# Autodesk Inventor assembly: Carriage_Assembly
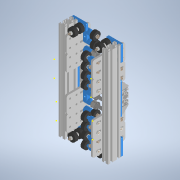
[picture p0: Inventor's stored thumbnail of the model, 180x180]
Saved by Autodesk Inventor 2021 (Build 250183000, 183)
## iProperties
Created: 2021-09-08
Part Number: Carriage_Assembly
Document SubType Name: Assembly
Designer: Jorian Brusind
Author: Jorian Brusind
## Documents named in this file (18)
- C:\Users\Jorian Brusind\Documents\GitHub\HyperRail\Inventor Files\Carriage_Assembly.iam
- C:\Users\Jorian Brusind\Documents\GitHub\HyperRail\Inventor Files\8020_Sets\IPT_20_Series\IPT_20_Series\20-2040_150mm.ipt
- C:\Users\Jorian Brusind\Documents\GitHub\HyperRail\Inventor Files\X_CarriageR_V2_0.iam
- C:\Users\Jorian Brusind\Documents\GitHub\HyperRail\Inventor Files\X_Carriage_V2_0.iam
- C:\Users\Jorian Brusind\Documents\GitHub\HyperRail\Inventor Files\8020_Sets\IPT_20_Series\Extra_20_Series\8020_14056m\14056_m.ipt
- C:\Users\Jorian Brusind\Documents\GitHub\HyperRail\Inventor Files\Buffer.iam
- C:\Users\Jorian Brusind\Documents\GitHub\HyperRail\Inventor Files\Metric Spacer_Standoffs\hex spacer standoff nut M5 L30.ipt
- C:\Users\Jorian Brusind\Documents\GitHub\HyperRail\Inventor Files\Carriage_Horizontal_Spacer.ipt
- C:\Users\Jorian Brusind\Documents\GitHub\HyperRail\Inventor Files\8020_Sets\IPT_20_Series\IPT_20_Series\20-2040_400mm.ipt
- C:\Users\Jorian Brusind\Documents\GitHub\HyperRail\Inventor Files\X_CarriageL_V2_1_Short.iam
- C:\Users\Jorian Brusind\Documents\GitHub\HyperRail\Inventor Files\X_CarriageR_V2_1_Short.iam
- C:\Users\Jorian Brusind\Documents\GitHub\HyperRail\Inventor Files\Buffer_L.iam
- C:\Users\Jorian Brusind\Documents\GitHub\HyperRail\Inventor Files\Metric bolt\Bolt M5 45mm.ipt
- C:\Users\Jorian Brusind\Documents\GitHub\HyperRail\Inventor Files\Metric bolt\Bolt M5 10mm.ipt
- C:\Users\Jorian Brusind\Documents\GitHub\HyperRail\Inventor Files\Metric nuts\Nut M5.ipt
- C:\Users\Jorian Brusind\Documents\GitHub\HyperRail\Inventor Files\X_CarriageL_V2_0_Short.iam
- C:\Users\Jorian Brusind\Documents\GitHub\HyperRail\Inventor Files\X_CarriageR_V2_0_Short.iam
- C:\Users\Jorian Brusind\Documents\GitHub\HyperRail\Inventor Files\din-508-t-slot-nut-t-nut-m4-m42-2.snapshot.3\STEPS\DIN 508, T-Slot Nut M5.ipt
## Components (98 placed, 17 different names)
1. 20-2040_150mm:1 — Mate:20, Mate:21, Mate:22, Mate:23, Mate:80, Flush:33, Flush:94, Flush:96, Flush:99, Flush:102, Flush:114
2. X_CarriageR_V2_0:1 [sub-assembly] — Mate:96, Flush:56, Flush:63, Flush:65, Flush:67, Mate:124, Mate:126, Mate:127, Mate:134, Mate:143, Mate:144, Mate:145, Mate:146, Mate:181, Mate:182, Mate:183, Mate:184, Flush:82, Flush:83, Flush:84, Mate:278
3. 14056_m:1 — Mate:21, Flush:26, Flush:38, Mate:167, Mate:168, Mate:169, Mate:170
4. 14056_m:2 — Mate:20, Flush:26, Mate:70, Flush:37, Flush:39, Mate:163, Mate:164, Mate:165, Mate:166
5. 14056_m:3 — Mate:22, Flush:13, Mate:155, Mate:156, Mate:157, Mate:158, Flush:115
6. 14056_m:4 — Mate:23, Flush:13, Mate:72, Mate:159, Mate:160, Mate:161, Mate:162, Flush:114, Flush:115, Flush:116
7. Buffer:2 [sub-assembly] — Mate:86, Flush:55, Mate:202, Mate:203, Mate:206, Mate:207, Flush:120
8. Buffer:3 [sub-assembly] — Flush:42, Mate:87, Mate:196, Mate:197, Mate:198, Mate:199, Flush:119, Mate:281
9. Carriage_Horizontal_Spacer:1 — Mate:72, Mate:79, Mate:80, Flush:116, Flush:117
10. Carriage_Horizontal_Spacer:2 — Mate:70, Mate:84, Flush:37, Flush:38, Flush:117
11. 20-2040_400mm:1 — Flush:30, Mate:75, Mate:76, Mate:79, Flush:33, Flush:36, Mate:86, Flush:55, Mate:111, Mate:112, Flush:59, Mate:140, Flush:71, Mate:216, Mate:217, Flush:97, Flush:98, Flush:100, Flush:101, Flush:103, Flush:104, Flush:118, Flush:120
12. 20-2040_400mm:2 — Flush:30, Flush:36, Mate:84, Flush:39, Flush:42, Mate:87, Mate:96, Mate:107, Mate:139, Flush:70, Mate:211, Mate:213, Mate:219, Mate:221, Mate:223, Flush:92, Flush:93, Flush:95, Flush:119, Flush:121
13. X_Carriage_V2_0:2 [sub-assembly] — Mate:107, Flush:63, Flush:64, Flush:65, Flush:67, Mate:130, Mate:131, Mate:138, Mate:152, Mate:153, Mate:154, Mate:179, Mate:180, Mate:185, Mate:186, Mate:191, Flush:81, Flush:90, Flush:91, Mate:277
14. X_CarriageL_V2_1_Short:1 [sub-assembly] — Mate:112, Flush:57, Flush:66, Mate:132, Mate:133, Mate:141, Mate:142, Mate:147, Mate:148, Flush:87, Mate:279
15. X_CarriageR_V2_1_Short:1 [sub-assembly] — Mate:111, Flush:56, Flush:57, Flush:59, Flush:64, Flush:66, Mate:135, Mate:136, Mate:137, Mate:149, Mate:150, Mate:151, Flush:86, Flush:112, Mate:276
16. hex spacer standoff nut M5 L30:1 — Mate:124, Mate:126, Mate:133
17. hex spacer standoff nut M5 L30:2 — Mate:130, Mate:135
18. hex spacer standoff nut M5 L30:3 — Mate:127, Mate:132, Mate:134
19. hex spacer standoff nut M5 L30:4 — Mate:131, Mate:136, Mate:137, Mate:138
20. Buffer_L:1 [sub-assembly] — Mate:139, Flush:70, Mate:192, Mate:193, Mate:194, Mate:195, Flush:121, Mate:280
21. Buffer_L:2 [sub-assembly] — Mate:140, Flush:71, Mate:200, Mate:201, Mate:204, Mate:205, Flush:118
22. Bolt M5 45mm:1 — Mate:142, Mate:148
23. Bolt M5 45mm:2 — Mate:141, Mate:147
24. Bolt M5 45mm:3 — Mate:143, Mate:145
25. Bolt M5 45mm:4 — Mate:144, Mate:146
26. Bolt M5 45mm:5 — Mate:150, Flush:73
27. Bolt M5 45mm:6 — Mate:149, Flush:73, Mate:151
28. Bolt M5 45mm:7 — Mate:153, Flush:74
29. Bolt M5 45mm:8 — Mate:152, Flush:74, Mate:154
30. Bolt M5 10mm:1 — Mate:156, Mate:158, Mate:231
31. Bolt M5 10mm:2 — Mate:155, Mate:157, Mate:232
32. Bolt M5 10mm:3 — Mate:164, Mate:165, Mate:227
33. Bolt M5 10mm:4 — Mate:168, Mate:169, Mate:222
34. Bolt M5 10mm:5 — Mate:163, Mate:166, Mate:228
35. Bolt M5 10mm:6 — Mate:167, Mate:170, Mate:224
36. Bolt M5 10mm:7 — Mate:160, Mate:162, Mate:234
37. Bolt M5 10mm:8 — Mate:159, Mate:161, Mate:233
38. Bolt M5 45mm:9 — Mate:181, Mate:183, Mate:187
39. Bolt M5 45mm:10 — Mate:182, Mate:184, Mate:188
40. Bolt M5 45mm:11 — Mate:179, Mate:185, Mate:189
41. Bolt M5 45mm:12 — Mate:180, Mate:186, Mate:190
42. Nut M5:5 — Mate:187, Flush:77
43. Nut M5:6 — Mate:188, Flush:76, Flush:77
44. Nut M5:7 — Mate:189, Flush:75
45. Nut M5:8 — Mate:190, Flush:75, Flush:76, Mate:191
46. Bolt M5 10mm:9 — Mate:192, Mate:195, Mate:225
47. Bolt M5 10mm:10 — Mate:193, Mate:194, Mate:226
48. Bolt M5 10mm:11 — Mate:202, Mate:206, Mate:230
49. Bolt M5 10mm:12 — Mate:201, Mate:205, Mate:236
50. Bolt M5 10mm:13 — Mate:203, Mate:207, Mate:229
51. Bolt M5 10mm:14 — Mate:200, Mate:204, Mate:235
52. Bolt M5 10mm:15 — Mate:197, Mate:198
53. Bolt M5 10mm:16 — Mate:196, Mate:199, Mate:220
54. X_Carriage_V2_0:3 [sub-assembly] — Mate:211, Flush:81, Flush:90, Flush:91, Mate:249, Mate:250, Mate:251, Mate:252, Mate:253, Mate:254, Mate:255, Mate:256, Mate:277, Mate:280
55. X_CarriageR_V2_0:2 [sub-assembly] — Flush:82, Mate:213, Flush:83, Flush:84, Mate:237, Mate:238, Mate:239, Mate:240, Mate:257, Mate:258, Mate:259, Mate:260, Mate:269, Mate:278, Mate:281
56. X_CarriageL_V2_0_Short:1 [sub-assembly] — Mate:217, Flush:87, Mate:241, Mate:242, Mate:243, Mate:244, Mate:270, Flush:113, Mate:279
57. X_CarriageR_V2_0_Short:1 [sub-assembly] — Flush:86, Mate:216, Mate:245, Mate:246, Mate:247, Mate:248, Flush:112, Flush:113, Mate:276
58. DIN 508, T-Slot Nut M5:1 — Mate:220, Mate:221
59. DIN 508, T-Slot Nut M5:2 — Mate:222, Mate:223
60. DIN 508, T-Slot Nut M5:3 — Mate:219
61. DIN 508, T-Slot Nut M5:4 — Mate:225, Flush:93
62. DIN 508, T-Slot Nut M5:5 — Mate:226, Flush:92
63. DIN 508, T-Slot Nut M5:6 — Mate:227, Flush:96
64. DIN 508, T-Slot Nut M5:7 — Mate:224, Flush:94
65. DIN 508, T-Slot Nut M5:8 — Mate:228, Flush:95
66. DIN 508, T-Slot Nut M5:10 — Mate:229, Flush:98
67. DIN 508, T-Slot Nut M5:11 — Mate:230, Flush:97
68. DIN 508, T-Slot Nut M5:12 — Mate:232, Flush:100
69. DIN 508, T-Slot Nut M5:13 — Mate:231, Flush:99
70. DIN 508, T-Slot Nut M5:14 — Mate:233, Flush:102
71. DIN 508, T-Slot Nut M5:15 — Mate:234, Flush:101
72. DIN 508, T-Slot Nut M5:16 — Mate:235, Flush:103
73. DIN 508, T-Slot Nut M5:17 — Mate:236, Flush:104
74. Bolt M5 45mm:13 — Mate:238, Mate:240, Mate:265
75. Bolt M5 45mm:14 — Mate:237, Mate:239, Mate:266
76. Bolt M5 45mm:15 — Mate:241, Mate:244, Mate:261
77. Bolt M5 45mm:16 — Mate:242, Mate:243, Mate:262
78. Bolt M5 45mm:17 — Mate:251, Mate:252, Mate:274
79. Bolt M5 45mm:18 — Mate:245, Mate:246, Mate:264, Mate:275
80. Bolt M5 45mm:19 — Mate:249, Mate:250, Mate:273
81. Bolt M5 45mm:20 — Mate:247, Mate:248, Mate:263
82. Bolt M5 45mm:21 — Mate:253, Mate:255, Mate:271
83. Bolt M5 45mm:22 — Mate:254, Mate:256, Mate:272
84. Bolt M5 45mm:23 — Mate:257, Mate:260, Mate:267
85. Bolt M5 45mm:24 — Mate:258, Mate:259, Mate:268
86. Nut M5:9 — Mate:264
87. Nut M5:10 — Mate:262, Flush:106, Mate:270
88. Nut M5:11 — Mate:266, Flush:105, Mate:269, Flush:110
89. Nut M5:12 — Mate:265, Flush:105
90. Nut M5:13 — Mate:267
91. Nut M5:14 — Mate:268, Flush:109
92. Nut M5:15 — Mate:263, Flush:111
93. Nut M5:16 — Mate:261, Flush:106
94. Nut M5:17 — Mate:274
95. Nut M5:18 — Mate:273, Flush:110
96. Nut M5:19 — Mate:271, Flush:109
97. Nut M5:20 — Mate:272
98. Nut M5:21 — Mate:275, Flush:111
## Relationships (220: Mate 157, Flush 63)
- Mate:20 (3 mm): 20-2040_150mm:1 ↔ 14056_m:2
- Mate:21 (3 mm): 20-2040_150mm:1 ↔ 14056_m:1
- Mate:22 (3 mm): 20-2040_150mm:1 ↔ 14056_m:3
- Mate:23 (3 mm): 20-2040_150mm:1 ↔ 14056_m:4
- Flush:13: 14056_m:3 ↔ 14056_m:4
- Flush:26: 14056_m:1 ↔ 14056_m:2
- Mate:70: 14056_m:2 ↔ Carriage_Horizontal_Spacer:2
- Mate:72: 14056_m:4 ↔ Carriage_Horizontal_Spacer:1
- Flush:30: 20-2040_400mm:1 ↔ 20-2040_400mm:2
- Mate:75: 20-2040_400mm:1
- Mate:76: 20-2040_400mm:1
- Mate:79: Carriage_Horizontal_Spacer:1 ↔ 20-2040_400mm:1
- Mate:80: 20-2040_150mm:1 ↔ Carriage_Horizontal_Spacer:1
- Flush:33: 20-2040_150mm:1 ↔ 20-2040_400mm:1
- Flush:36: 20-2040_400mm:1 ↔ 20-2040_400mm:2
- Mate:84: Carriage_Horizontal_Spacer:2 ↔ 20-2040_400mm:2
- Flush:37: 14056_m:2 ↔ Carriage_Horizontal_Spacer:2
- Flush:38: 14056_m:1 ↔ Carriage_Horizontal_Spacer:2
- Flush:39: 14056_m:2 ↔ 20-2040_400mm:2
- Mate:86: Buffer:2 ↔ 20-2040_400mm:1
- Flush:42: Buffer:3 ↔ 20-2040_400mm:2
- Mate:87: Buffer:3 ↔ 20-2040_400mm:2
- Mate:96: X_CarriageR_V2_0:1 ↔ 20-2040_400mm:2
- Flush:55: Buffer:2 ↔ 20-2040_400mm:1
- Mate:107: 20-2040_400mm:2 ↔ X_Carriage_V2_0:2
- Mate:111: 20-2040_400mm:1 ↔ X_CarriageR_V2_1_Short:1
- Flush:56: X_CarriageR_V2_0:1 ↔ X_CarriageR_V2_1_Short:1
- Mate:112: 20-2040_400mm:1 ↔ X_CarriageL_V2_1_Short:1
- Flush:57: X_CarriageL_V2_1_Short:1 ↔ X_CarriageR_V2_1_Short:1
- Flush:59: 20-2040_400mm:1 ↔ X_CarriageR_V2_1_Short:1
- Flush:63: X_CarriageR_V2_0:1 ↔ X_Carriage_V2_0:2
- Flush:64: X_Carriage_V2_0:2 ↔ X_CarriageR_V2_1_Short:1
- Flush:65: X_CarriageR_V2_0:1 ↔ X_Carriage_V2_0:2
- Flush:66: X_CarriageL_V2_1_Short:1 ↔ X_CarriageR_V2_1_Short:1
- Flush:67: X_CarriageR_V2_0:1 ↔ X_Carriage_V2_0:2
- Mate:124: X_CarriageR_V2_0:1 ↔ hex spacer standoff nut M5 L30:1
- Mate:126: X_CarriageR_V2_0:1 ↔ hex spacer standoff nut M5 L30:1
- Mate:127: X_CarriageR_V2_0:1 ↔ hex spacer standoff nut M5 L30:3
- Mate:130: X_Carriage_V2_0:2 ↔ hex spacer standoff nut M5 L30:2
- Mate:131: X_Carriage_V2_0:2 ↔ hex spacer standoff nut M5 L30:4
- Mate:132: X_CarriageL_V2_1_Short:1 ↔ hex spacer standoff nut M5 L30:3
- Mate:133: X_CarriageL_V2_1_Short:1 ↔ hex spacer standoff nut M5 L30:1
- Mate:134: X_CarriageR_V2_0:1 ↔ hex spacer standoff nut M5 L30:3
- Mate:135: X_CarriageR_V2_1_Short:1 ↔ hex spacer standoff nut M5 L30:2
- Mate:136: X_CarriageR_V2_1_Short:1 ↔ hex spacer standoff nut M5 L30:4
- Mate:137: X_CarriageR_V2_1_Short:1 ↔ hex spacer standoff nut M5 L30:4
- Mate:138: X_Carriage_V2_0:2 ↔ hex spacer standoff nut M5 L30:4
- Mate:139: 20-2040_400mm:2 ↔ Buffer_L:1
- Flush:70: 20-2040_400mm:2 ↔ Buffer_L:1
- Mate:140: 20-2040_400mm:1 ↔ Buffer_L:2
- Flush:71: 20-2040_400mm:1 ↔ Buffer_L:2
- Mate:141: X_CarriageL_V2_1_Short:1 ↔ Bolt M5 45mm:2
- Mate:142: X_CarriageL_V2_1_Short:1 ↔ Bolt M5 45mm:1
- Mate:143: X_CarriageR_V2_0:1 ↔ Bolt M5 45mm:3
- Mate:144: X_CarriageR_V2_0:1 ↔ Bolt M5 45mm:4
- Mate:145: X_CarriageR_V2_0:1 ↔ Bolt M5 45mm:3
- Mate:146: X_CarriageR_V2_0:1 ↔ Bolt M5 45mm:4
- Mate:147: X_CarriageL_V2_1_Short:1 ↔ Bolt M5 45mm:2
- Mate:148: X_CarriageL_V2_1_Short:1 ↔ Bolt M5 45mm:1
- Mate:149: X_CarriageR_V2_1_Short:1 ↔ Bolt M5 45mm:6
- Mate:150: X_CarriageR_V2_1_Short:1 ↔ Bolt M5 45mm:5
- Flush:73: Bolt M5 45mm:5 ↔ Bolt M5 45mm:6
- Mate:151: X_CarriageR_V2_1_Short:1 ↔ Bolt M5 45mm:6
- Mate:152: X_Carriage_V2_0:2 ↔ Bolt M5 45mm:8
- Mate:153: X_Carriage_V2_0:2 ↔ Bolt M5 45mm:7
- Flush:74: Bolt M5 45mm:7 ↔ Bolt M5 45mm:8
- Mate:154: X_Carriage_V2_0:2 ↔ Bolt M5 45mm:8
- Mate:155: 14056_m:3 ↔ Bolt M5 10mm:2
- Mate:156: 14056_m:3 ↔ Bolt M5 10mm:1
- Mate:157: 14056_m:3 ↔ Bolt M5 10mm:2
- Mate:158: 14056_m:3 ↔ Bolt M5 10mm:1
- Mate:159: 14056_m:4 ↔ Bolt M5 10mm:8
- Mate:160: 14056_m:4 ↔ Bolt M5 10mm:7
- Mate:161: 14056_m:4 ↔ Bolt M5 10mm:8
- Mate:162: 14056_m:4 ↔ Bolt M5 10mm:7
- Mate:163: 14056_m:2 ↔ Bolt M5 10mm:5
- Mate:164: 14056_m:2 ↔ Bolt M5 10mm:3
- Mate:165: 14056_m:2 ↔ Bolt M5 10mm:3
- Mate:166: 14056_m:2 ↔ Bolt M5 10mm:5
- Mate:167: 14056_m:1 ↔ Bolt M5 10mm:6
- Mate:168: 14056_m:1 ↔ Bolt M5 10mm:4
- Mate:169: 14056_m:1 ↔ Bolt M5 10mm:4
- Mate:170: 14056_m:1 ↔ Bolt M5 10mm:6
- Mate:179: X_Carriage_V2_0:2 ↔ Bolt M5 45mm:11
- Mate:180: X_Carriage_V2_0:2 ↔ Bolt M5 45mm:12
- Mate:181: X_CarriageR_V2_0:1 ↔ Bolt M5 45mm:9
- Mate:182: X_CarriageR_V2_0:1 ↔ Bolt M5 45mm:10
- Mate:183: X_CarriageR_V2_0:1 ↔ Bolt M5 45mm:9
- Mate:184: X_CarriageR_V2_0:1 ↔ Bolt M5 45mm:10
- Mate:185: X_Carriage_V2_0:2 ↔ Bolt M5 45mm:11
- Mate:186: X_Carriage_V2_0:2 ↔ Bolt M5 45mm:12
- Mate:187: Bolt M5 45mm:9 ↔ Nut M5:5
- Mate:188: Bolt M5 45mm:10 ↔ Nut M5:6
- Mate:189: Bolt M5 45mm:11 ↔ Nut M5:7
- Mate:190: Bolt M5 45mm:12 ↔ Nut M5:8
- Flush:75: Nut M5:7 ↔ Nut M5:8
- Flush:76: Nut M5:6 ↔ Nut M5:8
- Flush:77: Nut M5:5 ↔ Nut M5:6
- Mate:191: X_Carriage_V2_0:2 ↔ Nut M5:8
- Mate:192: Buffer_L:1 ↔ Bolt M5 10mm:9
- Mate:193: Buffer_L:1 ↔ Bolt M5 10mm:10
- Mate:194: Buffer_L:1 ↔ Bolt M5 10mm:10
- Mate:195: Buffer_L:1 ↔ Bolt M5 10mm:9
- Mate:196: Buffer:3 ↔ Bolt M5 10mm:16
- Mate:197: Buffer:3 ↔ Bolt M5 10mm:15
- Mate:198: Buffer:3 ↔ Bolt M5 10mm:15
- Mate:199: Buffer:3 ↔ Bolt M5 10mm:16
- Mate:200: Buffer_L:2 ↔ Bolt M5 10mm:14
- Mate:201: Buffer_L:2 ↔ Bolt M5 10mm:12
- Mate:202: Buffer:2 ↔ Bolt M5 10mm:11
- Mate:203: Buffer:2 ↔ Bolt M5 10mm:13
- Mate:204: Buffer_L:2 ↔ Bolt M5 10mm:14
- Mate:205: Buffer_L:2 ↔ Bolt M5 10mm:12
- Mate:206: Buffer:2 ↔ Bolt M5 10mm:11
- Mate:207: Buffer:2 ↔ Bolt M5 10mm:13
- Mate:211: 20-2040_400mm:2 ↔ X_Carriage_V2_0:3
- Flush:81: X_Carriage_V2_0:2 ↔ X_Carriage_V2_0:3
- Flush:82: X_CarriageR_V2_0:1 ↔ X_CarriageR_V2_0:2
- Mate:213: 20-2040_400mm:2 ↔ X_CarriageR_V2_0:2
- Flush:83: X_CarriageR_V2_0:1 ↔ X_CarriageR_V2_0:2
- Flush:84: X_CarriageR_V2_0:1 ↔ X_CarriageR_V2_0:2
- Flush:86: X_CarriageR_V2_1_Short:1 ↔ X_CarriageR_V2_0_Short:1
- Mate:216: 20-2040_400mm:1 ↔ X_CarriageR_V2_0_Short:1
- Mate:217: 20-2040_400mm:1 ↔ X_CarriageL_V2_0_Short:1
- Flush:87: X_CarriageL_V2_1_Short:1 ↔ X_CarriageL_V2_0_Short:1
- Flush:90: X_Carriage_V2_0:2 ↔ X_Carriage_V2_0:3
- Flush:91: X_Carriage_V2_0:2 ↔ X_Carriage_V2_0:3
- Mate:219: 20-2040_400mm:2 ↔ DIN 508, T-Slot Nut M5:3
- Mate:220: Bolt M5 10mm:16 ↔ DIN 508, T-Slot Nut M5:1
- Mate:221: 20-2040_400mm:2 ↔ DIN 508, T-Slot Nut M5:1
- Mate:222: Bolt M5 10mm:4 ↔ DIN 508, T-Slot Nut M5:2
- Mate:223: 20-2040_400mm:2 ↔ DIN 508, T-Slot Nut M5:2
- Mate:224: Bolt M5 10mm:6 ↔ DIN 508, T-Slot Nut M5:7
- Mate:225: Bolt M5 10mm:9 ↔ DIN 508, T-Slot Nut M5:4
- Mate:226: Bolt M5 10mm:10 ↔ DIN 508, T-Slot Nut M5:5
- Flush:92: 20-2040_400mm:2 ↔ DIN 508, T-Slot Nut M5:5
- Flush:93: 20-2040_400mm:2 ↔ DIN 508, T-Slot Nut M5:4
- Flush:94: 20-2040_150mm:1 ↔ DIN 508, T-Slot Nut M5:7
- Mate:227: Bolt M5 10mm:3 ↔ DIN 508, T-Slot Nut M5:6
- Mate:228: Bolt M5 10mm:5 ↔ DIN 508, T-Slot Nut M5:8
- Flush:95: 20-2040_400mm:2 ↔ DIN 508, T-Slot Nut M5:8
- Flush:96: 20-2040_150mm:1 ↔ DIN 508, T-Slot Nut M5:6
- Mate:229: Bolt M5 10mm:13 ↔ DIN 508, T-Slot Nut M5:10
- Mate:230: Bolt M5 10mm:11 ↔ DIN 508, T-Slot Nut M5:11
- Flush:97: 20-2040_400mm:1 ↔ DIN 508, T-Slot Nut M5:11
- Flush:98: 20-2040_400mm:1 ↔ DIN 508, T-Slot Nut M5:10
- Mate:231: Bolt M5 10mm:1 ↔ DIN 508, T-Slot Nut M5:13
- Mate:232: Bolt M5 10mm:2 ↔ DIN 508, T-Slot Nut M5:12
- Flush:99: 20-2040_150mm:1 ↔ DIN 508, T-Slot Nut M5:13
- Flush:100: 20-2040_400mm:1 ↔ DIN 508, T-Slot Nut M5:12
- Mate:233: Bolt M5 10mm:8 ↔ DIN 508, T-Slot Nut M5:14
- Mate:234: Bolt M5 10mm:7 ↔ DIN 508, T-Slot Nut M5:15
- Flush:101: 20-2040_400mm:1 ↔ DIN 508, T-Slot Nut M5:15
- Flush:102: 20-2040_150mm:1 ↔ DIN 508, T-Slot Nut M5:14
- Mate:235: Bolt M5 10mm:14 ↔ DIN 508, T-Slot Nut M5:16
- Flush:103: 20-2040_400mm:1 ↔ DIN 508, T-Slot Nut M5:16
- Mate:236: Bolt M5 10mm:12 ↔ DIN 508, T-Slot Nut M5:17
- Flush:104: 20-2040_400mm:1 ↔ DIN 508, T-Slot Nut M5:17
- Mate:237: X_CarriageR_V2_0:2 ↔ Bolt M5 45mm:14
- Mate:238: X_CarriageR_V2_0:2 ↔ Bolt M5 45mm:13
- Mate:239: X_CarriageR_V2_0:2 ↔ Bolt M5 45mm:14
- Mate:240: X_CarriageR_V2_0:2 ↔ Bolt M5 45mm:13
- Mate:241: X_CarriageL_V2_0_Short:1 ↔ Bolt M5 45mm:15
- Mate:242: X_CarriageL_V2_0_Short:1 ↔ Bolt M5 45mm:16
- Mate:243: X_CarriageL_V2_0_Short:1 ↔ Bolt M5 45mm:16
- Mate:244: X_CarriageL_V2_0_Short:1 ↔ Bolt M5 45mm:15
- Mate:245: X_CarriageR_V2_0_Short:1 ↔ Bolt M5 45mm:18
- Mate:246: X_CarriageR_V2_0_Short:1 ↔ Bolt M5 45mm:18
- Mate:247: X_CarriageR_V2_0_Short:1 ↔ Bolt M5 45mm:20
- Mate:248: X_CarriageR_V2_0_Short:1 ↔ Bolt M5 45mm:20
- Mate:249: X_Carriage_V2_0:3 ↔ Bolt M5 45mm:19
- Mate:250: X_Carriage_V2_0:3 ↔ Bolt M5 45mm:19
- Mate:251: X_Carriage_V2_0:3 ↔ Bolt M5 45mm:17
- Mate:252: X_Carriage_V2_0:3 ↔ Bolt M5 45mm:17
- Mate:253: X_Carriage_V2_0:3 ↔ Bolt M5 45mm:21
- Mate:254: X_Carriage_V2_0:3 ↔ Bolt M5 45mm:22
- Mate:255: X_Carriage_V2_0:3 ↔ Bolt M5 45mm:21
- Mate:256: X_Carriage_V2_0:3 ↔ Bolt M5 45mm:22
- Mate:257: X_CarriageR_V2_0:2 ↔ Bolt M5 45mm:23
- Mate:258: X_CarriageR_V2_0:2 ↔ Bolt M5 45mm:24
- Mate:259: X_CarriageR_V2_0:2 ↔ Bolt M5 45mm:24
- Mate:260: X_CarriageR_V2_0:2 ↔ Bolt M5 45mm:23
- Mate:261: Bolt M5 45mm:15 ↔ Nut M5:16
- Mate:262: Bolt M5 45mm:16 ↔ Nut M5:10
- Mate:263: Bolt M5 45mm:20 ↔ Nut M5:15
- Mate:264: Bolt M5 45mm:18 ↔ Nut M5:9
- Mate:265: Bolt M5 45mm:13 ↔ Nut M5:12
- Mate:266: Bolt M5 45mm:14 ↔ Nut M5:11
- Mate:267: Bolt M5 45mm:23 ↔ Nut M5:13
- Mate:268: Bolt M5 45mm:24 ↔ Nut M5:14
- Flush:105: Nut M5:11 ↔ Nut M5:12
- Mate:269: X_CarriageR_V2_0:2 ↔ Nut M5:11
- Flush:106: Nut M5:10 ↔ Nut M5:16
- Mate:270: X_CarriageL_V2_0_Short:1 ↔ Nut M5:10
- [Flush]: Nut M5:17 ↔ Nut M5:18
- [Flush]: Nut M5:19 ↔ Nut M5:20
- Mate:271: Bolt M5 45mm:21 ↔ Nut M5:19
- Mate:272: Bolt M5 45mm:22 ↔ Nut M5:20
- Flush:109: Nut M5:14 ↔ Nut M5:19
- Mate:273: Bolt M5 45mm:19 ↔ Nut M5:18
- Mate:274: Bolt M5 45mm:17 ↔ Nut M5:17
- Flush:110: Nut M5:11 ↔ Nut M5:18
- Mate:275: Bolt M5 45mm:18 ↔ Nut M5:21
- Flush:111: Nut M5:15 ↔ Nut M5:21
- Flush:112: X_CarriageR_V2_1_Short:1 ↔ X_CarriageR_V2_0_Short:1
- Flush:113: X_CarriageL_V2_0_Short:1 ↔ X_CarriageR_V2_0_Short:1
- Flush:114: 20-2040_150mm:1 ↔ 14056_m:4
- Flush:115: 14056_m:3 ↔ 14056_m:4
- Flush:116 (-7 mm): 14056_m:4 ↔ Carriage_Horizontal_Spacer:1
- Flush:117: Carriage_Horizontal_Spacer:1 ↔ Carriage_Horizontal_Spacer:2
- Mate:276: X_CarriageR_V2_1_Short:1 ↔ X_CarriageR_V2_0_Short:1
- Mate:277: X_Carriage_V2_0:2 ↔ X_Carriage_V2_0:3
- Mate:278: X_CarriageR_V2_0:1 ↔ X_CarriageR_V2_0:2
- Mate:279: X_CarriageL_V2_1_Short:1 ↔ X_CarriageL_V2_0_Short:1
- Flush:118: 20-2040_400mm:1 ↔ Buffer_L:2
- Flush:119: Buffer:3 ↔ 20-2040_400mm:2
- Flush:120: Buffer:2 ↔ 20-2040_400mm:1
- Flush:121: 20-2040_400mm:2 ↔ Buffer_L:1
- Mate:280: Buffer_L:1 ↔ X_Carriage_V2_0:3
- Mate:281: Buffer:3 ↔ X_CarriageR_V2_0:2
## Named parameters: d390_d388 = 0 mm, d391_d388 = 0 mm
